# Autodesk Inventor assembly: Ensemble tout
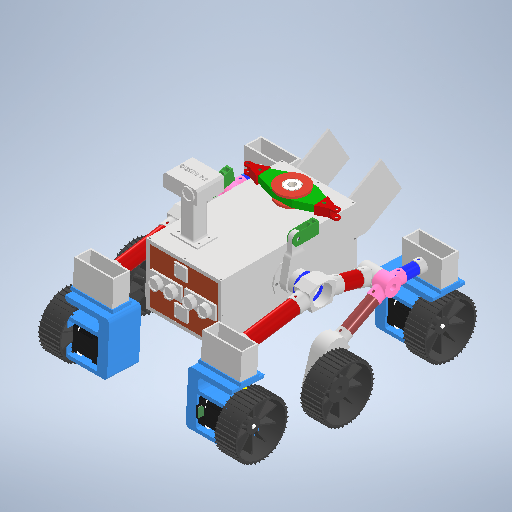
[picture p0: Inventor's stored thumbnail of the model, 512x512]
Saved by Autodesk Inventor 2026.2 (Build 302298010, 298A)
## iProperties
Created: 2026-03-16
Part Number: Ensemble tout
Document SubType Name: Assembly
Designer: genon
Author: genon
## Documents named in this file (31)
- C:\Users\genon\Documents\Henallux Passerelle\Projet de conception\Cassini T-X\Inventor\Ensemble tout.iam
- C:\Users\genon\Documents\Henallux Passerelle\Projet de conception\Cassini T-X\Inventor\Ensemble_Boite_chassis.iam
- C:\Users\genon\Documents\Henallux Passerelle\Projet de conception\Cassini T-X\Inventor\Suspension\Ensemble_Relier_suspension.iam
- C:\Users\genon\Documents\Henallux Passerelle\Projet de conception\Cassini T-X\Inventor\Suspension\tube vers bogie.ipt
- C:\Users\genon\Documents\Henallux Passerelle\Projet de conception\Cassini T-X\Inventor\Suspension\bielle sup.ipt
- C:\Users\genon\Documents\Henallux Passerelle\Projet de conception\Cassini T-X\Inventor\Suspension\bielle côté 0.ipt
- C:\Users\genon\Documents\Henallux Passerelle\Projet de conception\Cassini T-X\Inventor\Suspension\bièlle côté.ipt
- C:\Users\genon\Documents\Henallux Passerelle\Projet de conception\Cassini T-X\Inventor\Suspension\Rolling v2.ipt
- C:\Users\genon\Documents\Henallux Passerelle\Projet de conception\Cassini T-X\Inventor\Suspension\bielle côté 2.ipt
- C:\Users\genon\Documents\Henallux Passerelle\Projet de conception\Cassini T-X\Inventor\Suspension\bielle côté 3.ipt
- C:\Users\genon\Documents\Henallux Passerelle\Projet de conception\Cassini T-X\Inventor\Suspension\tubelong_rocker.ipt
- C:\Users\genon\Documents\Henallux Passerelle\Projet de conception\Cassini T-X\Inventor\Suspension\Attache servomoteur.ipt
- C:\Users\genon\Documents\Henallux Passerelle\Projet de conception\Cassini T-X\Inventor\Suspension\Attache moteur.ipt
- C:\Users\genon\Documents\Henallux Passerelle\Projet de conception\Cassini T-X\Inventor\Suspension\bielle rocker.ipt
- C:\Users\genon\Documents\Henallux Passerelle\Projet de conception\Cassini T-X\Inventor\Suspension\bielle rocker2.ipt
- C:\Users\genon\Documents\Henallux Passerelle\Projet de conception\Cassini T-X\Inventor\Suspension\tube des bogies.ipt
- C:\Users\genon\Documents\Henallux Passerelle\Projet de conception\Cassini T-X\Inventor\Suspension\bielle roue milieu.ipt
- C:\Users\genon\Documents\Henallux Passerelle\Projet de conception\Cassini T-X\Inventor\Suspension\Attache servomoteur_bogie.ipt
- C:\Users\genon\Documents\Henallux Passerelle\Projet de conception\Cassini T-X\Inventor\Suspension\mr_105_2rs.ipt
- C:\Users\genon\Documents\Henallux Passerelle\Projet de conception\Cassini T-X\Inventor\Composants\Stepper Motor\Stepper Motor\Stepper Motor.ipt
- C:\Users\genon\Documents\Henallux Passerelle\Projet de conception\Cassini T-X\Inventor\Suspension\Attache moteur côté rocker.ipt
- C:\Users\genon\Documents\Henallux Passerelle\Projet de conception\Cassini T-X\Inventor\Suspension\roulement 22mm.ipt
- C:\Users\genon\Documents\Henallux Passerelle\Projet de conception\Cassini T-X\Inventor\Suspension\Roue.ipt
- C:\Users\genon\Documents\Henallux Passerelle\Projet de conception\Cassini T-X\Inventor\Suspension\Roue libre.ipt
- C:\Users\genon\Documents\Henallux Passerelle\Projet de conception\Cassini T-X\Inventor\Suspension\bielle roue milieu autre côté.ipt
- C:\Users\genon\Documents\Henallux Passerelle\Projet de conception\Cassini T-X\Inventor\Composants\US HC-SR04.ipt
- C:\Users\genon\Documents\Henallux Passerelle\Projet de conception\Cassini T-X\Inventor\Composants\TOF - VL6180X Fermion SEN0427.ipt
- C:\Users\genon\Documents\Henallux Passerelle\Projet de conception\Cassini T-X\Inventor\Suspension\tube vers roue libre.ipt
- C:\Users\genon\Documents\Henallux Passerelle\Projet de conception\Cassini T-X\Inventor\Accessoires\Caméra.ipt
- C:\Users\genon\Documents\Henallux Passerelle\Projet de conception\Cassini T-X\Inventor\Accessoires\Bras caméra.ipt
- C:\Users\genon\Documents\Henallux Passerelle\Projet de conception\Cassini T-X\Inventor\Accessoires\autour hélice.ipt
## Components (62 placed, 30 different names)
1. Ensemble_Boite_chassis:1 [sub-assembly] — Placage:2, Placage:15, Placage:16, Placage:63, Placage:64, Cylindrique:15, Placage:137, Placage:138, Placage:139, Placage:142, Placage:143, Placage:144, Placage:160, Placage:161, Placage:162, Placage:167, Placage:168, Placage:169
2. Ensemble_Relier_suspension:1 [sub-assembly] — Placage:2, Cylindrique:15
3. bielle sup:1 — Cylindrique:19, Placage:129
4. bielle côté 0:1 — Placage:15, Placage:16, Cylindrique:2, Placage:19, Placage:138
5. bièlle côté:1 — Cylindrique:1, Placage:18, Placage:19, Placage:20, Placage:21, Placage:22, Cylindrique:3, Placage:128, Cylindrique:18, Placage:129
6. Rolling v2:1 — Cylindrique:1, Placage:18, Cylindrique:2
7. bielle côté 2:1 — Placage:20, Placage:21, Placage:22, Placage:23, Placage:149, Placage:150, Placage:151
8. Rolling v2:2 — Cylindrique:3, Placage:23
9. tubelong_rocker:1 — Placage:30, Placage:31, Placage:152, Placage:153
10. Attache servomoteur:1 — Placage:30, Placage:31, Placage:57, Placage:58, Placage:59
11. tube vers bogie:3 — Placage:37, Placage:38, Placage:154, Placage:155
12. bielle rocker:1 — Placage:37, Placage:38, Placage:40, Cylindrique:9, Placage:97
13. bielle rocker2:1 — Placage:40, Placage:43, Placage:44, Cylindrique:10, Placage:145, Placage:146
14. tube des bogies:1 — Placage:43, Placage:44, Placage:47, Placage:48
15. bielle roue milieu:1
16. Attache servomoteur_bogie:1 — Placage:47, Placage:48, Placage:49, Placage:50, Placage:51
17. Attache moteur:3 — Placage:49, Placage:50, Placage:51, Placage:99, Placage:100, Affleurement:1
18. mr_105_2rs:1 — Placage:128, Cylindrique:18, Cylindrique:19
19. Stepper Motor:1 — Placage:93, Placage:94, Placage:95, Placage:99, Placage:100, Affleurement:1
20. Attache moteur côté rocker:1 — Placage:57, Placage:58, Placage:59, Placage:108, Affleurement:3, Placage:140
21. bielle roue milieu:2 — Placage:102, Placage:103, Placage:147, Placage:148
22. bièlle côté:2 — Placage:65, Placage:66, Placage:67, Placage:68, Placage:69, Placage:70, Placage:126, Cylindrique:16, Placage:127
23. bielle côté 0:2 — Placage:63, Placage:64, Cylindrique:7, Placage:67, Placage:68, Placage:139
24. roulement 22mm:1 — Placage:65, Placage:66, Cylindrique:7
25. bielle côté 2:2 — Placage:69, Placage:70, Cylindrique:8, Placage:71, Placage:72, Placage:73
26. roulement 22mm:2 — Cylindrique:8, Placage:71
27. bielle côté 3:3 — Placage:72, Placage:73, Placage:74, Placage:75, Placage:78, Placage:79
28. tubelong_rocker:2 — Placage:74, Placage:75, Placage:76, Placage:77
29. Attache servomoteur:2 — Placage:76, Placage:77, Placage:133, Placage:134, Placage:135
30. tube vers bogie:4 — Placage:78, Placage:79, Placage:80, Placage:81
31. bielle rocker:2 — Placage:80, Placage:81, Placage:83, Cylindrique:11, Placage:98
32. roulement 22mm:3 — Cylindrique:11, Placage:98, Cylindrique:12
33. bielle rocker2:2 — Placage:83, Placage:86, Placage:87, Cylindrique:12, Placage:156, Placage:157
34. tube des bogies:4 — Placage:86, Placage:87, Placage:88, Placage:89
35. Attache servomoteur_bogie:2 — Placage:88, Placage:89, Placage:130, Placage:131, Placage:132
36. Attache moteur côté rocker:2 — Affleurement:2, Placage:107, Placage:133, Placage:134, Placage:135, Placage:141
37. Roue:1 — Placage:114, Placage:115, Placage:116
38. Roue:2 — Placage:93, Placage:94, Placage:95
39. roulement 22mm:4 — Cylindrique:9, Placage:97, Cylindrique:10
40. Roue libre:1 — Cylindrique:13, Placage:101, Placage:102, Placage:103
41. roulement 22mm:5 — Cylindrique:13, Placage:101
42. bielle roue milieu autre côté:1 — Placage:121, Placage:122, Placage:158, Placage:159
43. Stepper Motor:2 — Affleurement:2, Placage:107, Placage:117, Placage:118, Placage:119, Placage:141
44. Stepper Motor:3 — Placage:108, Affleurement:3, Placage:123, Placage:124, Placage:125, Placage:140
45. Attache moteur:4 — Placage:112, Placage:113, Affleurement:4, Placage:130, Placage:131, Placage:132
46. Stepper Motor:4 — Placage:112, Placage:113, Affleurement:4, Placage:114, Placage:115, Placage:116
47. Roue libre:2 — Cylindrique:14, Placage:120, Placage:121, Placage:122
48. Roue:3 — Placage:117, Placage:118, Placage:119
49. roulement 22mm:6 — Cylindrique:14, Placage:120
50. Roue:4 — Placage:123, Placage:124, Placage:125
51. bielle sup:2 — Cylindrique:17, Placage:127
52. mr_105_2rs:2 — Placage:126, Cylindrique:16, Cylindrique:17
53. US HC-SR04:1 — Placage:144
54. US HC-SR04:2 — Placage:137
55. TOF - VL6180X Fermion SEN0427:1 — Placage:143
56. TOF - VL6180X Fermion SEN0427:2 — Placage:142
57. tube vers roue libre:1 — Placage:145, Placage:146, Placage:147, Placage:148
58. bielle côté 3:4 — Placage:149, Placage:150, Placage:151, Placage:152, Placage:153, Placage:154, Placage:155
59. tube vers roue libre:2 — Placage:156, Placage:157, Placage:158, Placage:159
60. Bras caméra:1 — Placage:160, Placage:161, Placage:162, Placage:163, Placage:164, Placage:165
61. Caméra:1 — Placage:163, Placage:164, Placage:165
62. autour hélice:1 — Placage:167, Placage:168, Placage:169
## Relationships (136: Mate 116, CylindricalJoint 16, Flush 4)
- Placage:2 [Mate]: Ensemble_Boite_chassis:1 ↔ Ensemble_Relier_suspension:1
- Placage:15 [Mate]: Ensemble_Boite_chassis:1 ↔ bielle côté 0:1
- Placage:16 [Mate]: Ensemble_Boite_chassis:1 ↔ bielle côté 0:1
- Cylindrique:1: bièlle côté:1 ↔ Rolling v2:1
- Placage:18 [Mate]: bièlle côté:1 ↔ Rolling v2:1
- Cylindrique:2: bielle côté 0:1 ↔ Rolling v2:1
- Placage:19 [Mate]: bielle côté 0:1 ↔ bièlle côté:1
- Placage:20 [Mate]: bièlle côté:1 ↔ bielle côté 2:1
- Placage:21 [Mate]: bièlle côté:1 ↔ bielle côté 2:1
- Placage:22 [Mate]: bièlle côté:1 ↔ bielle côté 2:1
- Cylindrique:3: bièlle côté:1 ↔ Rolling v2:2
- Placage:23 [Mate]: bielle côté 2:1 ↔ Rolling v2:2
- Placage:30 [Mate]: tubelong_rocker:1 ↔ Attache servomoteur:1
- Placage:31 [Mate]: tubelong_rocker:1 ↔ Attache servomoteur:1
- Placage:37 [Mate]: tube vers bogie:3 ↔ bielle rocker:1
- Placage:38 [Mate]: tube vers bogie:3 ↔ bielle rocker:1
- Placage:40 [Mate]: bielle rocker:1 ↔ bielle rocker2:1
- Placage:43 [Mate]: bielle rocker2:1 ↔ tube des bogies:1
- Placage:44 [Mate]: bielle rocker2:1 ↔ tube des bogies:1
- Placage:47 [Mate]: tube des bogies:1 ↔ Attache servomoteur_bogie:1
- Placage:48 [Mate]: tube des bogies:1 ↔ Attache servomoteur_bogie:1
- Placage:49 [Mate]: Attache servomoteur_bogie:1 ↔ Attache moteur:3
- Placage:50 [Mate]: Attache servomoteur_bogie:1 ↔ Attache moteur:3
- Placage:51 [Mate]: Attache servomoteur_bogie:1 ↔ Attache moteur:3
- Placage:57 [Mate]: Attache servomoteur:1 ↔ Attache moteur côté rocker:1
- Placage:58 [Mate]: Attache servomoteur:1 ↔ Attache moteur côté rocker:1
- Placage:59 [Mate]: Attache servomoteur:1 ↔ Attache moteur côté rocker:1
- Placage:63 [Mate]: Ensemble_Boite_chassis:1 ↔ bielle côté 0:2
- Placage:64 [Mate]: Ensemble_Boite_chassis:1 ↔ bielle côté 0:2
- Placage:65 [Mate]: bièlle côté:2 ↔ roulement 22mm:1
- Placage:66 [Mate]: bièlle côté:2 ↔ roulement 22mm:1
- Cylindrique:7: bielle côté 0:2 ↔ roulement 22mm:1
- Placage:67 [Mate]: bièlle côté:2 ↔ bielle côté 0:2
- Placage:68 [Mate]: bièlle côté:2 ↔ bielle côté 0:2
- Placage:69 [Mate]: bièlle côté:2 ↔ bielle côté 2:2
- Placage:70 [Mate]: bièlle côté:2 ↔ bielle côté 2:2
- Cylindrique:8: bielle côté 2:2 ↔ roulement 22mm:2
- Placage:71 [Mate]: bielle côté 2:2 ↔ roulement 22mm:2
- Placage:72 [Mate]: bielle côté 2:2 ↔ bielle côté 3:3
- Placage:73 [Mate]: bielle côté 2:2 ↔ bielle côté 3:3
- Placage:74 [Mate]: bielle côté 3:3 ↔ tubelong_rocker:2
- Placage:75 [Mate]: bielle côté 3:3 ↔ tubelong_rocker:2
- Placage:76 [Mate]: tubelong_rocker:2 ↔ Attache servomoteur:2
- Placage:77 [Mate]: tubelong_rocker:2 ↔ Attache servomoteur:2
- Placage:78 [Mate]: bielle côté 3:3 ↔ tube vers bogie:4
- Placage:79 [Mate]: bielle côté 3:3 ↔ tube vers bogie:4
- Placage:80 [Mate]: tube vers bogie:4 ↔ bielle rocker:2
- Placage:81 [Mate]: tube vers bogie:4 ↔ bielle rocker:2
- Placage:83 [Mate]: bielle rocker:2 ↔ bielle rocker2:2
- Placage:86 [Mate]: bielle rocker2:2 ↔ tube des bogies:4
- Placage:87 [Mate]: bielle rocker2:2 ↔ tube des bogies:4
- Placage:88 [Mate]: tube des bogies:4 ↔ Attache servomoteur_bogie:2
- Placage:89 [Mate]: tube des bogies:4 ↔ Attache servomoteur_bogie:2
- Placage:93 [Mate]: Stepper Motor:1 ↔ Roue:2
- Placage:94 [Mate]: Stepper Motor:1 ↔ Roue:2
- Placage:95 [Mate]: Stepper Motor:1 ↔ Roue:2
- Cylindrique:9: bielle rocker:1 ↔ roulement 22mm:4
- Placage:97 [Mate]: bielle rocker:1 ↔ roulement 22mm:4
- Cylindrique:10: bielle rocker2:1 ↔ roulement 22mm:4
- Cylindrique:11: bielle rocker:2 ↔ roulement 22mm:3
- Placage:98 [Mate]: bielle rocker:2 ↔ roulement 22mm:3
- Cylindrique:12: roulement 22mm:3 ↔ bielle rocker2:2
- Placage:99 [Mate]: Attache moteur:3 ↔ Stepper Motor:1
- Placage:100 [Mate]: Attache moteur:3 ↔ Stepper Motor:1
- Affleurement:1 [Flush] (2.588 mm): Attache moteur:3 ↔ Stepper Motor:1
- Cylindrique:13: Roue libre:1 ↔ roulement 22mm:5
- Placage:101 [Mate]: Roue libre:1 ↔ roulement 22mm:5
- Placage:102 [Mate]: bielle roue milieu:2 ↔ Roue libre:1
- Placage:103 [Mate]: bielle roue milieu:2 ↔ Roue libre:1
- Affleurement:2 [Flush] (2.388 mm): Attache moteur côté rocker:2 ↔ Stepper Motor:2
- Placage:107 [Mate]: Attache moteur côté rocker:2 ↔ Stepper Motor:2
- Placage:108 [Mate]: Attache moteur côté rocker:1 ↔ Stepper Motor:3
- Affleurement:3 [Flush] (2.388 mm): Attache moteur côté rocker:1 ↔ Stepper Motor:3
- Placage:112 [Mate]: Attache moteur:4 ↔ Stepper Motor:4
- Placage:113 [Mate]: Attache moteur:4 ↔ Stepper Motor:4
- Affleurement:4 [Flush] (2.388 mm): Attache moteur:4 ↔ Stepper Motor:4
- Placage:114 [Mate]: Roue:1 ↔ Stepper Motor:4
- Placage:115 [Mate]: Roue:1 ↔ Stepper Motor:4
- Placage:116 [Mate]: Roue:1 ↔ Stepper Motor:4
- Placage:117 [Mate]: Stepper Motor:2 ↔ Roue:3
- Placage:118 [Mate]: Stepper Motor:2 ↔ Roue:3
- Placage:119 [Mate]: Stepper Motor:2 ↔ Roue:3
- Cylindrique:14: Roue libre:2 ↔ roulement 22mm:6
- Placage:120 [Mate]: Roue libre:2 ↔ roulement 22mm:6
- Placage:121 [Mate]: bielle roue milieu autre côté:1 ↔ Roue libre:2
- Placage:122 [Mate]: bielle roue milieu autre côté:1 ↔ Roue libre:2
- Placage:123 [Mate]: Stepper Motor:3 ↔ Roue:4
- Placage:124 [Mate]: Stepper Motor:3 ↔ Roue:4
- Placage:125 [Mate]: Stepper Motor:3 ↔ Roue:4
- Cylindrique:15: Ensemble_Boite_chassis:1 ↔ Ensemble_Relier_suspension:1
- Placage:126 [Mate]: bièlle côté:2 ↔ mr_105_2rs:2
- Cylindrique:16: bièlle côté:2 ↔ mr_105_2rs:2
- Cylindrique:17: bielle sup:2 ↔ mr_105_2rs:2
- Placage:127 [Mate]: bièlle côté:2 ↔ bielle sup:2
- Placage:128 [Mate]: bièlle côté:1 ↔ mr_105_2rs:1
- Cylindrique:18: bièlle côté:1 ↔ mr_105_2rs:1
- Cylindrique:19: bielle sup:1 ↔ mr_105_2rs:1
- Placage:129 [Mate]: bielle sup:1 ↔ bièlle côté:1
- Placage:130 [Mate]: Attache servomoteur_bogie:2 ↔ Attache moteur:4
- Placage:131 [Mate]: Attache servomoteur_bogie:2 ↔ Attache moteur:4
- Placage:132 [Mate]: Attache servomoteur_bogie:2 ↔ Attache moteur:4
- Placage:133 [Mate]: Attache servomoteur:2 ↔ Attache moteur côté rocker:2
- Placage:134 [Mate]: Attache servomoteur:2 ↔ Attache moteur côté rocker:2
- Placage:135 [Mate]: Attache servomoteur:2 ↔ Attache moteur côté rocker:2
- Placage:137 [Mate]: Ensemble_Boite_chassis:1 ↔ US HC-SR04:2
- Placage:138 [Mate]: Ensemble_Boite_chassis:1 ↔ bielle côté 0:1
- Placage:139 [Mate]: Ensemble_Boite_chassis:1 ↔ bielle côté 0:2
- Placage:140 [Mate]: Attache moteur côté rocker:1 ↔ Stepper Motor:3
- Placage:141 [Mate]: Attache moteur côté rocker:2 ↔ Stepper Motor:2
- Placage:142 [Mate]: Ensemble_Boite_chassis:1 ↔ TOF - VL6180X Fermion SEN0427:2
- Placage:143 [Mate]: Ensemble_Boite_chassis:1 ↔ TOF - VL6180X Fermion SEN0427:1
- Placage:144 [Mate]: Ensemble_Boite_chassis:1 ↔ US HC-SR04:1
- Placage:145 [Mate]: bielle rocker2:1 ↔ tube vers roue libre:1
- Placage:146 [Mate]: bielle rocker2:1 ↔ tube vers roue libre:1
- Placage:147 [Mate]: bielle roue milieu:2 ↔ tube vers roue libre:1
- Placage:148 [Mate]: bielle roue milieu:2 ↔ tube vers roue libre:1
- Placage:149 [Mate]: bielle côté 2:1 ↔ bielle côté 3:4
- Placage:150 [Mate]: bielle côté 2:1 ↔ bielle côté 3:4
- Placage:151 [Mate]: bielle côté 2:1 ↔ bielle côté 3:4
- Placage:152 [Mate]: tubelong_rocker:1 ↔ bielle côté 3:4
- Placage:153 [Mate]: tubelong_rocker:1 ↔ bielle côté 3:4
- Placage:154 [Mate]: tube vers bogie:3 ↔ bielle côté 3:4
- Placage:155 [Mate]: tube vers bogie:3 ↔ bielle côté 3:4
- Placage:156 [Mate]: bielle rocker2:2 ↔ tube vers roue libre:2
- Placage:157 [Mate]: bielle rocker2:2 ↔ tube vers roue libre:2
- Placage:158 [Mate]: bielle roue milieu autre côté:1 ↔ tube vers roue libre:2
- Placage:159 [Mate]: bielle roue milieu autre côté:1 ↔ tube vers roue libre:2
- Placage:160 [Mate]: Ensemble_Boite_chassis:1 ↔ Bras caméra:1
- Placage:161 [Mate]: Ensemble_Boite_chassis:1 ↔ Bras caméra:1
- Placage:162 [Mate]: Ensemble_Boite_chassis:1 ↔ Bras caméra:1
- Placage:163 [Mate]: Bras caméra:1 ↔ Caméra:1
- Placage:164 [Mate]: Bras caméra:1 ↔ Caméra:1
- Placage:165 [Mate]: Bras caméra:1 ↔ Caméra:1
- Placage:167 [Mate]: Ensemble_Boite_chassis:1 ↔ autour hélice:1
- Placage:168 [Mate]: Ensemble_Boite_chassis:1 ↔ autour hélice:1
- Placage:169 [Mate]: Ensemble_Boite_chassis:1 ↔ autour hélice:1
